# Autodesk Inventor assembly: Full_Assembly
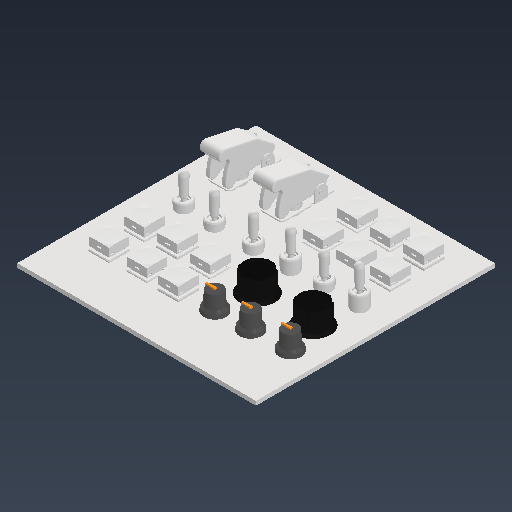
[picture p0: Inventor's stored thumbnail of the model, 512x512]
Saved by Autodesk Inventor 2025.3 (Build 293356000, 356)
## iProperties
Created: 2025-09-08
Part Number: Full_Assembly
Document SubType Name: Assembly
Designer: tolga
Author: tolga
## Documents named in this file (8)
- C:\Users\tolga\Documents\Repositories\Personal Projects\Sim-Control-Panel-v1.0\CAD\Full_Assembly.iam
- C:\Users\tolga\Documents\Repositories\Personal Projects\Sim-Control-Panel-v1.0\CAD\3rd_Party_Parts\Lighted_Buttons\Lighted_Buttons.iam
- C:\Users\tolga\Documents\Repositories\Personal Projects\Sim-Control-Panel-v1.0\CAD\3rd_Party_Parts\On-On Switch.ipt
- C:\Users\tolga\Documents\Repositories\Personal Projects\Sim-Control-Panel-v1.0\CAD\3rd_Party_Parts\Momentary Switch.ipt
- C:\Users\tolga\Documents\Repositories\Personal Projects\Sim-Control-Panel-v1.0\CAD\3rd_Party_Parts\Encoder_Knob.ipt
- C:\Users\tolga\Documents\Repositories\Personal Projects\Sim-Control-Panel-v1.0\CAD\3rd_Party_Parts\Potentiometer Knob.ipt
- C:\Users\tolga\Documents\Repositories\Personal Projects\Sim-Control-Panel-v1.0\CAD\3rd_Party_Parts\Switch Guard.ipt
- C:\Users\tolga\Documents\Repositories\Personal Projects\Sim-Control-Panel-v1.0\CAD\Faceplate.ipt
## Components (28 placed, 7 different names)
1. Lighted_Buttons:1 [sub-assembly]
2. Lighted_Buttons:2 [sub-assembly]
3. Lighted_Buttons:3 [sub-assembly]
4. Lighted_Buttons:4 [sub-assembly]
5. Lighted_Buttons:5 [sub-assembly]
6. Lighted_Buttons:6 [sub-assembly]
7. Lighted_Buttons:7 [sub-assembly]
8. Lighted_Buttons:8 [sub-assembly]
9. Lighted_Buttons:9 [sub-assembly]
10. Lighted_Buttons:10 [sub-assembly]
11. Lighted_Buttons:11 [sub-assembly]
12. Lighted_Buttons:12 [sub-assembly]
13. On-On Switch:1 — Insert:1
14. Momentary Switch:1
15. Momentary Switch:2
16. Momentary Switch:3
17. Encoder_Knob:1
18. Encoder_Knob:2
19. Momentary Switch:4
20. Momentary Switch:5
21. Momentary Switch:6
22. Potentiometer Knob:1
23. Potentiometer Knob:2
24. Potentiometer Knob:3
25. Switch Guard:1 — Insert:1
26. On-On Switch:2
27. Switch Guard:3
28. Faceplate:1
## Relationships (2: Insert 2)
- Insert:1 (5 mm): On-On Switch:1 ↔ Switch Guard:1
- [Insert] (5 mm): On-On Switch:2 ↔ Switch Guard:3
## Named parameters: d1_d0 = 5 mm
